# Autodesk Inventor assembly: journal finaliam
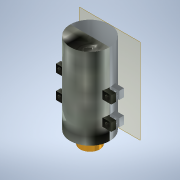
[picture p0: Inventor's stored thumbnail of the model, 180x180]
Saved by Autodesk Inventor 2021 (Build 250183000, 183)
## iProperties
Created: 2022-10-30
Part Number: journal finaliam
Document SubType Name: Assembly
Designer: Eng Ahmed khaled
Author: Eng Ahmed khaled
## Documents named in this file (5)
- F:\senior 2 1st\heat\project\journal finaliam.iam
- F:\senior 2 1st\heat\project\5972K246_Ball Bearing.ipt
- F:\senior 2 1st\heat\project\CUP_lower_part.ipt
- F:\senior 2 1st\heat\project\CUP_upper_part.ipt
- F:\senior 2 1st\heat\project\Shaftipt.ipt
## Components (5 placed, 4 different names)
1. 5972K246_Ball Bearing:1 — Mate:1, Mate:2, Mate:5, Mate:6
2. CUP_lower_part:1 — Mate:5, Mate:6, Mate:7, Mate:8, Mate:9, Mate:10
3. CUP_upper_part:1 — Mate:7, Mate:8, Mate:9, Mate:10
4. Shaftipt:1 — Mate:1, Mate:2, Mate:3, Mate:4
5. 5972K246_Ball Bearing:2 — Mate:3, Mate:4
## Relationships (10: Mate 10)
- Mate:1: 5972K246_Ball Bearing:1 ↔ Shaftipt:1
- Mate:2: 5972K246_Ball Bearing:1 ↔ Shaftipt:1
- Mate:3: Shaftipt:1 ↔ 5972K246_Ball Bearing:2
- Mate:4: Shaftipt:1 ↔ 5972K246_Ball Bearing:2
- Mate:5: 5972K246_Ball Bearing:1 ↔ CUP_lower_part:1
- Mate:6: 5972K246_Ball Bearing:1 ↔ CUP_lower_part:1
- Mate:7: CUP_lower_part:1 ↔ CUP_upper_part:1
- Mate:8: CUP_lower_part:1 ↔ CUP_upper_part:1
- Mate:9: CUP_lower_part:1 ↔ CUP_upper_part:1
- Mate:10: CUP_lower_part:1 ↔ CUP_upper_part:1
